# Autodesk Inventor assembly: CP96SDB32-50-M9P(0_0_0)
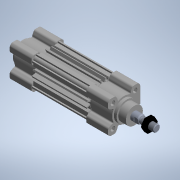
[picture p0: Inventor's stored thumbnail of the model, 180x180]
Saved by Autodesk Inventor 2021 (Build 250183000, 183)
## iProperties
Category: PARTsolutions
Company: SMC
Part Number: CP96SDB32-50-M9P(0_0_0)
Catalog Web Link: www.cadenas.de
Description: CP96S/CP96SD-ISO Cylinder:Standard Double Acting,Single/Double Rod
Vendor: SMC
Document SubType Name: Assembly
Designer: partserver
Manufacturer: SMC
Mass: 212.172 g
Surface Area: 658.778 cm^2
Volume: 212.172 cm^3
Density: 1 g/cm^3
PSOL_IDENT_0: {$CADENAS_DATA\23d-libs\smc_jp\actuator\standard_air_cylinder\cp96_c96\cp96_asmtab.prj},280 {VTYP=3D
PSOL_IDENT_1: },{STYP=ASSTAB},{NB=CP96SDB32-50-M9P(0_0_0)},{LINA=CP96SDB32-50-M9P},{NN=CP96S/CP96SD},{DATE=05.07.2
PSOL_IDENT_2: 021 01:48:16},{GEOMDATE=24.12.2018 05:26:10},{VERSION=},{LINEID=10},{WBVAR=MAGNET,AUTOSWITCH,LEAD,NU
PSOL_IDENT_3: MBER,STROKE,POS,ROD,BOOT,STOP,ATEX,OMSC,THREAD},{WBNUMERIC=STROKE,POS}  {NB=CP96SDB32-50-M9P(0_0_0)}
PSOL_IDENT_4: ,{LINA=CP96SDB32-50-M9P},{KT=DUMMY},{BORE=32},{MOUNT=(B) Basic},{MOUNTX=B},{MAGNET=D},{AUTOSWITCH=-M
PSOL_IDENT_5: 9P},{AUTOSWITCHX='','(-) Without autoswitch','-M9N','M9N','-M9P','M9P','-M9B','M9B','-M9NW','M9NW','
PSOL_IDENT_6: -M9PW','M9PW','-M9BW','M9BW','-M9NA','M9NA','-M9PA','M9PA','-M9BA','M9BA','-A96','A96','-A93','A93','
PSOL_IDENT_7: -A90','A90'},{SWITCH=B},{LEAD=},{LEADX='','(-) 0.5 m','M','(M) 1 m','L','(L) 3 m','Z','(Z) 5 m'},{NU
PSOL_IDENT_8: MBER=},{NUMBERX='', '(-) 2 pcs', 'S', '(S) 1 pc'},{STROKE=50},{STDSTROKE=25,50,80,100,125,160,200,25
PSOL_IDENT_9: 0,320,400,500},{STROKEX=25,50,80,100,125,160,200,250,320,400,500},{SMINX=15},{SMAX=2000},{SMAXX=2000
PSOL_IDENT_10: },{POS=0},{ROD=},{RODX='','(-) Single rod','W','(W) Double rod'},{BOOT=},{BOOTX='','(-) Without boot'
PSOL_IDENT_11: ,'J','(J) Nylon tarpaulin (one end)','K','(K) Heat resistant tarpaulin (one end)'},{STOP=0},{STOPX='
PSOL_IDENT_12: 0','Standard stroke','1','Manufacturable stroke'},{COM=-},{ATEX=},{ATEXX='','N/A'},{OMSC=},{OMSCX=''
PSOL_IDENT_13: ,'(-) Without order','-XC4','(-XC4) With heavy duty scraper','-XC7','(-XC7) Tie-rod, cushion valve,
PSOL_IDENT_14: tie-rod nut, etc. Made of stainless steel','-XC18','(-XC18) Port thread type NPT','-XC22','(-XC22) F
PSOL_IDENT_15: luororubber seals','-XC35','(-XC35) With coil scraper','-XC68','(-XC68) Made of stainless steel (Wit
PSOL_IDENT_16: h hard chrome plated piston rod)'},{THREAD=0},{ORDER=CP96SDB32-50-M9P},{A=22},{B=30},{D=12},{EE=G 1/
PSOL_IDENT_17: 8},{PL=13.0},{RT=M6x1},{L12=6.0},{KK=M10x1.25},{SW=10},{G=32.0},{BG=16},{L8=94},{VD=4},{VA=4},{WA=4.
PSOL_IDENT_18: 0},{WB=7.0},{WH=26},{ZZ=146},{ZY=190},{E=47},{R=32.5},{L2=15},{L9=4},{H=48},{E1=48},{TR=32},{AH=32},
PSOL_IDENT_19: {AO=10},{AT=4.5},{AB=7.0},{SA=142},{XA=144},{TM=50},{TL=12},{TD=12},{UW=49},{L1=17},{XV=73.0},{Z=95.
PSOL_IDENT_20: 0},{RF=32},{TF=64},{FB=7},{E2=50},{UF=79},{W=16},{MF=10},{ZF=130},{UB=45},{CB=26},{EW=26-0.2/-0.6},{
PSOL_IDENT_21: CD=10},{L=12},{MR=9.5},{XD=142},{EB=65},{A1=10.5},{A2=6.5},{B1=8.0},{B2=4.0},{AA=10.5},{BB=8.0},{PPA
PSOL_IDENT_22: TH=cp96/assembly/cp96_asmsbl.prj},{MODEL=CP96SDB32-50-M9P},{NENN=CP96SB32}
NB: CP96SDB32-50-M9P(0_0_0)
NN: CP96S/CP96SD
NT: ISO Cylinder:Standard Double Acting,Single/Double Rod
NBSYN: $ORDER.($POS._$STOP._$THREAD.)
LINA: CP96SDB32-50-M9P
CATALOG: SMC (JP
ROWDESC: CP96SB32
BORE: 32
MOUNT: (B) Basic
MAGNET: (D) With magnet
AUTOSWITCH: M9P Solid state-General-Grommet-Indicator light:Yes-3 wire(PNP)-In line
LEAD: (-) 0.5 m
NUMBER: (-) 2 pcs
STROKE: 50
POS: 0
ROD: (-) Single rod
BOOT: (-) Without boot
STOP: Standard stroke
COM: -
ATEX: N/A
OMSC: (-) Without order
THREAD: on
SUPPLIER: SMC
ARTICLENO: CP96SDB32-50-M9P(0_0_0)
BOMINFO: CP96SDB32-50-M9P
CREATOR: CADENAS GmbH
Title: CP96SDB32-50-M9P
Author: Cadenas PARTsolutions
Comments: ISO Cylinder:Standard Double Acting,Single/Double Rod
## Documents named in this file (5)
- C:\Users\Nelson\Github\Proyecto_APM\Inventor_Corte\AIS2021\CP96SDB32-50-M9P(0_0_0).iam
- C:\Users\Nelson\Github\Proyecto_APM\Inventor_Corte\AIS2021\CP96S32-50(0)_BODY.ipt
- C:\Users\Nelson\Github\Proyecto_APM\Inventor_Corte\AIS2021\CP96-M9P_SW.ipt
- C:\Users\Nelson\Github\Proyecto_APM\Inventor_Corte\AIS2021\CP96S32-50_ROD.ipt
- C:\Users\Nelson\Github\Proyecto_APM\Inventor_Corte\AIS2021\C96S32_NUT.ipt
## Components (5 placed, 4 different names)
1. CP96S32-50(0)_BODY:1 — Flush:2, Mate:3, Flush:3, Mate:4
2. CP96-M9P_SW:1 — Flush:3, Mate:4, Mate:5
3. CP96S32-50_ROD:1 — Flush:1, Flush:4, Mate:5
4. C96S32_NUT:1
5. CP96-M9P_SW:2 — Flush:2, Mate:3, Flush:4
## Relationships (7: Flush 4, Mate 3)
- Flush:1 (-50 mm): CP96S32-50_ROD:1
- Flush:2: CP96S32-50(0)_BODY:1 ↔ CP96-M9P_SW:2
- Mate:3 (0.1 mm): CP96S32-50(0)_BODY:1 ↔ CP96-M9P_SW:2
- Flush:3: CP96S32-50(0)_BODY:1 ↔ CP96-M9P_SW:1
- Mate:4 (0.1 mm): CP96S32-50(0)_BODY:1 ↔ CP96-M9P_SW:1
- Flush:4 (-2 mm): CP96S32-50_ROD:1 ↔ CP96-M9P_SW:2
- Mate:5 (-21.2183 mm): CP96-M9P_SW:1 ↔ CP96S32-50_ROD:1
